# Autodesk Inventor assembly: Kornylak Wheel with Hub
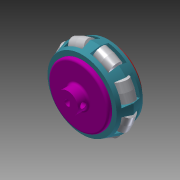
[picture p0: Inventor's stored thumbnail of the model, 180x180]
Saved by Autodesk Inventor 2014 (Build 180170000, 170)
## iProperties
Created: 2014-02-14
Part Number: Kornylak Wheel with Hub
Document SubType Name: Assembly
Designer: Spooner
Author: Spooner
## Documents named in this file (4)
- C:\Users\Spooner\Documents\Inventor\FerretBall Robot\3Pod\Inventor 2014 Files\Kornylak Wheel with Hub.iam
- C:\Users\Spooner\Documents\Inventor\FerretBall Robot\3Pod\Inventor 2014 Files\Kornylak Wheel.iam
- C:\Users\Spooner\Documents\Inventor\FerretBall Robot\3Pod\Inventor 2014 Files\Kornylak Wheel Hub - Motor Side.ipt
- C:\Users\Spooner\Documents\Inventor\FerretBall Robot\3Pod\Inventor 2014 Files\Kornylak Wheel Hub - Out Side.ipt
## Components (3 placed, 3 different names)
1. Kornylak Wheel:1 [sub-assembly] — Insert:1, Insert:2
2. Kornylak Wheel Hub - Motor Side:1 — Insert:2
3. Kornylak Wheel Hub - Out Side:1 — Insert:1
## Relationships (2: Insert 2)
- Insert:1: Kornylak Wheel:1 ↔ Kornylak Wheel Hub - Out Side:1
- Insert:2: Kornylak Wheel:1 ↔ Kornylak Wheel Hub - Motor Side:1
